# Autodesk Inventor assembly: PCB Stack Concept V03 01
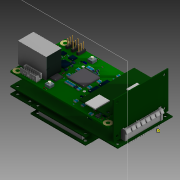
[picture p0: Inventor's stored thumbnail of the model, 180x180]
Saved by Autodesk Inventor 2013 (Build 170138000, 138)
## iProperties
Created: 2014-04-13
Part Number: PCB Stack Concept V03 01
Document SubType Name: Assembly
Designer: spichelh
Author: spichelh
## Documents named in this file (30)
- C:\Users\spichelh\Documents\GitHub\beta-hardware\Enclosure\Version 002\PCB Stack Concept V03 01.iam
- C:\Users\spichelh\Documents\GitHub\beta-hardware\Enclosure\Version 002\Enclosure-Backplate01.ipt
- C:\Users\spichelh\Documents\GitHub\beta-hardware\Enclosure\Version 002\KAC12040.ipt
- C:\Users\spichelh\Documents\GitHub\beta-hardware\Enclosure\Version 002\IRGlass.ipt
- C:\Users\spichelh\Documents\GitHub\beta-hardware\Enclosure\Version 002\Cooler.ipt
- C:\Users\spichelh\Documents\GitHub\beta-hardware\Enclosure\Version 002\Nikon Mount 02.ipt
- C:\Users\spichelh\Documents\GitHub\beta-hardware\Enclosure\Version 002\IOModulePlate01.ipt
- C:\Users\spichelh\Documents\GitHub\beta-hardware\Enclosure\Version 002\PCBModuleLeft01.ipt
- C:\Users\spichelh\Documents\GitHub\beta-hardware\Enclosure\Version 002\IOModulePlate02.ipt
- C:\Users\spichelh\Documents\GitHub\beta-hardware\Enclosure\Version 002\IOModulePlate03.ipt
- C:\Users\spichelh\Documents\GitHub\beta-hardware\Enclosure\Version 002\PCBModuleRight01.ipt
- C:\Users\spichelh\Documents\GitHub\beta-hardware\Enclosure\Version 002\LensBase02.ipt
- C:\Users\spichelh\Documents\GitHub\beta-hardware\Enclosure\Version 002\HexSaver01.ipt
- C:\Users\spichelh\Documents\GitHub\beta-hardware\Enclosure\Version 002\Enclosure03.ipt
- C:\Users\spichelh\Documents\Inventor\Content Center Files\R2013\en-US\ANSI B18.3.1M(1)\ANSI B18.3.1M - M2,5x0,45 x 16(2).ipt
- C:\Users\spichelh\Documents\Inventor\Content Center Files\R2013\en-US\ANSI B18.3.1M(1)\ANSI B18.3.1M - M2,5x0,45 x 35(2).ipt
- C:\Users\spichelh\Documents\GitHub\beta-hardware\Enclosure\Version 002\LensBaseTop01.ipt
- C:\Users\spichelh\Documents\Inventor\Content Center Files\R2013\en-US\ANSI B18.6.3(00)\ANSI B18.6.3 - 3-48 UNC - 0,25(32).ipt
- C:\Users\spichelh\Documents\GitHub\beta-hardware\Enclosure\Version 002\Unmate01.ipt
- C:\Users\spichelh\Documents\GitHub\beta-hardware\Enclosure\Version 002\Parallella.ipt
- C:\Users\spichelh\Documents\GitHub\beta-hardware\Enclosure\Version 002\SFE-Host01.ipt
- C:\Users\spichelh\Documents\GitHub\beta-hardware\Enclosure\Version 002\SFE-ProcessingBoard01.ipt
- C:\Users\spichelh\Documents\GitHub\beta-hardware\Enclosure\Version 002\CMV12000.ipt
- C:\Users\spichelh\Documents\GitHub\beta-hardware\Enclosure\Version 002\Enclosure-Backplate-Variant02.ipt
- C:\Users\spichelh\Documents\GitHub\beta-hardware\Enclosure\Version 002\PCBModuleLeft02.ipt
- C:\Users\spichelh\Documents\GitHub\beta-hardware\Enclosure\Version 002\BetaBoard01.ipt
- C:\Users\spichelh\Documents\GitHub\beta-hardware\Enclosure\Version 002\Imported Components\Zynq_Z010_uZed_F_Prod\Zynq_Z010_uZed_F_Prod.ipt
- C:\Users\spichelh\Documents\GitHub\beta-hardware\Enclosure\Version 002\Imported Components\c-5-1612163-2-h-3d\c-5-1612163-2-h-3d.ipt
- C:\Users\spichelh\Documents\GitHub\beta-hardware\Enclosure\Version 002\HidhSpeedIOShield01.ipt
- C:\Users\spichelh\Documents\GitHub\beta-hardware\Enclosure\Version 002\AddonPCB01.ipt
## Components (42 placed, 29 different names)
1. Enclosure03:1 — Flush:26, Mate:33, Mate:34, Mate:38, Flush:40, Mate:39, Insert:9, Insert:10, Insert:11, Insert:13, Insert:14, Insert:27, Insert:28, Insert:29, Mate:70, Mate:71, Flush:46, Flush:47
2. Enclosure-Backplate01:1 — Mate:38, Flush:40, Mate:75
3. KAC12040:1 — Mate:72
4. IRGlass:1 — Mate:50, Mate:51, Mate:52
5. Cooler:1 — Mate:35, Flush:43, Flush:44, Mate:67, Mate:68, Mate:69
6. Nikon Mount 02:1 — Mate:31, Mate:32, Insert:3, Mate:50, Mate:51, Mate:52, Insert:18, Insert:19, Insert:20, Insert:21
7. LensBase02:1 — Mate:31, Mate:32, Flush:26, Mate:33, Mate:34, Insert:3, Mate:35, Flush:43, Flush:44, Flush:45
8. IOModulePlate01:1 — Insert:13, Insert:14
9. PCBModuleLeft01:1
10. PCBModuleRight01:1
11. IOModulePlate02:1 — Insert:11
12. IOModulePlate03:1 — Insert:9, Insert:10
13. HexSaver01:1
14. HexSaver01:2
15. HexSaver01:3
16. HexSaver01:4
17. Broached Socket Head Cap Screw - Metric M2,5x0,45 x 16:1 — Insert:18
18. Broached Socket Head Cap Screw - Metric M2,5x0,45 x 16:2 — Insert:19
19. Broached Socket Head Cap Screw - Metric M2,5x0,45 x 16:3 — Insert:20
20. Broached Socket Head Cap Screw - Metric M2,5x0,45 x 16:4 — Insert:21
21. LensBaseTop01:1 — Flush:45, Mate:53, Mate:54, Mate:67, Mate:68, Mate:69
22. Cross Recessed 100° Flat Countersunk Head Machine Screw - Type I - Inch 3-48 UNC x 0,25:2 — Mate:53
23. Cross Recessed 100° Flat Countersunk Head Machine Screw - Type I - Inch 3-48 UNC x 0,25:1 — Mate:54
24. Broached Socket Head Cap Screw - Metric M2,5x0,45 x 35:5 — Mate:55, Mate:70, Mate:71
25. Broached Socket Head Cap Screw - Metric M2,5x0,45 x 35:6 — Insert:27, Mate:59
26. Broached Socket Head Cap Screw - Metric M2,5x0,45 x 35:7 — Insert:28, Mate:66
27. Broached Socket Head Cap Screw - Metric M2,5x0,45 x 35:8 — Insert:29, Mate:57
28. Unmate01:1 — Mate:55
29. Unmate01:2 — Mate:57
30. Unmate01:3 — Mate:59
31. Unmate01:4 — Mate:66
32. Parallella:1
33. SFE-Host01:1 — Mate:72, Mate:73, Flush:48, Flush:49, Mate:76, Flush:50, Flush:51, Flush:78
34. SFE-ProcessingBoard01:1 — Mate:73, Flush:48, Flush:49, Mate:77, Flush:85
35. CMV12000:1 — Mate:76, Flush:50, Flush:51
36. Enclosure-Backplate-Variant02:1 — Mate:75, Flush:46, Flush:47
37. PCBModuleLeft02:1 — Flush:52, Flush:79, Mate:79
38. BetaBoard01:1 — Mate:77, Flush:52, Flush:78, Flush:79, Mate:78, Flush:82, Flush:83, Mate:79, Flush:85, Flush:86, Flush:87, Mate:80, Flush:88
39. Zynq_Z010_uZed_F_Prod:1 — Flush:86, Flush:87, Mate:80, Flush:91, Mate:83, Flush:92
40. c-5-1612163-2-h-3d:1 — Mate:78, Flush:82, Flush:83, Mate:81, Mate:82
41. HidhSpeedIOShield01:1 — Mate:81, Flush:88, Mate:82
42. AddonPCB01:1 — Flush:91, Mate:83, Flush:92
## Relationships (67: Mate 32, Flush 22, Insert 13)
- Mate:31: Nikon Mount 02:1 ↔ LensBase02:1
- Mate:32: Nikon Mount 02:1 ↔ LensBase02:1
- Flush:26: Enclosure03:1 ↔ LensBase02:1
- Mate:33: Enclosure03:1 ↔ LensBase02:1
- Mate:34: Enclosure03:1 ↔ LensBase02:1
- Insert:3: Nikon Mount 02:1 ↔ LensBase02:1
- Mate:35: Cooler:1 ↔ LensBase02:1
- Mate:38 (3 mm): Enclosure03:1 ↔ Enclosure-Backplate01:1
- Flush:40: Enclosure03:1 ↔ Enclosure-Backplate01:1
- Mate:39: Enclosure03:1
- Insert:9: Enclosure03:1 ↔ IOModulePlate03:1
- Insert:10: Enclosure03:1 ↔ IOModulePlate03:1
- Insert:11: Enclosure03:1 ↔ IOModulePlate02:1
- Insert:13: Enclosure03:1 ↔ IOModulePlate01:1
- Insert:14: Enclosure03:1 ↔ IOModulePlate01:1
- Mate:50: IRGlass:1 ↔ Nikon Mount 02:1
- Mate:51 (0.5 mm): IRGlass:1 ↔ Nikon Mount 02:1
- Mate:52 (0.5 mm): IRGlass:1 ↔ Nikon Mount 02:1
- Flush:43: Cooler:1 ↔ LensBase02:1
- Flush:44: Cooler:1 ↔ LensBase02:1
- Flush:45: LensBase02:1 ↔ LensBaseTop01:1
- Mate:55: Broached Socket Head Cap Screw - Metric M2,5x0,45 x 35:5 ↔ Unmate01:1
- Mate:57: Broached Socket Head Cap Screw - Metric M2,5x0,45 x 35:8 ↔ Unmate01:2
- Mate:59: Broached Socket Head Cap Screw - Metric M2,5x0,45 x 35:6 ↔ Unmate01:3
- Mate:66: Broached Socket Head Cap Screw - Metric M2,5x0,45 x 35:7 ↔ Unmate01:4
- Mate:67: Cooler:1 ↔ LensBaseTop01:1
- Mate:68: Cooler:1 ↔ LensBaseTop01:1
- Mate:69: Cooler:1 ↔ LensBaseTop01:1
- Mate:70: Enclosure03:1 ↔ Broached Socket Head Cap Screw - Metric M2,5x0,45 x 35:5
- Mate:71: Enclosure03:1 ↔ Broached Socket Head Cap Screw - Metric M2,5x0,45 x 35:5
- Mate:72: KAC12040:1 ↔ SFE-Host01:1
- Mate:73: SFE-Host01:1 ↔ SFE-ProcessingBoard01:1
- Mate:75 (10 mm): Enclosure-Backplate01:1 ↔ Enclosure-Backplate-Variant02:1
- Flush:46: Enclosure03:1 ↔ Enclosure-Backplate-Variant02:1
- Flush:47: Enclosure03:1 ↔ Enclosure-Backplate-Variant02:1
- Flush:48: SFE-Host01:1 ↔ SFE-ProcessingBoard01:1
- Flush:49: SFE-Host01:1 ↔ SFE-ProcessingBoard01:1
- Mate:76 (3 mm): SFE-Host01:1 ↔ CMV12000:1
- Flush:50 (5 mm): SFE-Host01:1 ↔ CMV12000:1
- Flush:51 (11.75 mm): SFE-Host01:1 ↔ CMV12000:1
- Mate:77: SFE-ProcessingBoard01:1 ↔ BetaBoard01:1
- Flush:52: PCBModuleLeft02:1 ↔ BetaBoard01:1
- Flush:78: SFE-Host01:1 ↔ BetaBoard01:1
- Flush:79: PCBModuleLeft02:1 ↔ BetaBoard01:1
- Mate:78: BetaBoard01:1 ↔ c-5-1612163-2-h-3d:1
- Flush:82 (8.5 mm): BetaBoard01:1 ↔ c-5-1612163-2-h-3d:1
- Flush:83 (2 mm): BetaBoard01:1 ↔ c-5-1612163-2-h-3d:1
- Mate:79 (6 mm): PCBModuleLeft02:1 ↔ BetaBoard01:1
- Flush:85 (-21 mm): SFE-ProcessingBoard01:1 ↔ BetaBoard01:1
- Flush:86: BetaBoard01:1 ↔ Zynq_Z010_uZed_F_Prod:1
- Flush:87: BetaBoard01:1 ↔ Zynq_Z010_uZed_F_Prod:1
- Mate:80 (12 mm): BetaBoard01:1 ↔ Zynq_Z010_uZed_F_Prod:1
- Mate:81: c-5-1612163-2-h-3d:1 ↔ HidhSpeedIOShield01:1
- Flush:88: BetaBoard01:1 ↔ HidhSpeedIOShield01:1
- Mate:82: c-5-1612163-2-h-3d:1 ↔ HidhSpeedIOShield01:1
- Flush:91: Zynq_Z010_uZed_F_Prod:1 ↔ AddonPCB01:1
- Mate:83: Zynq_Z010_uZed_F_Prod:1 ↔ AddonPCB01:1
- Flush:92: Zynq_Z010_uZed_F_Prod:1 ↔ AddonPCB01:1
- Insert:18: Nikon Mount 02:1 ↔ Broached Socket Head Cap Screw - Metric M2,5x0,45 x 16:1
- Insert:19: Nikon Mount 02:1 ↔ Broached Socket Head Cap Screw - Metric M2,5x0,45 x 16:2
- Insert:20: Nikon Mount 02:1 ↔ Broached Socket Head Cap Screw - Metric M2,5x0,45 x 16:3
- Insert:21: Nikon Mount 02:1 ↔ Broached Socket Head Cap Screw - Metric M2,5x0,45 x 16:4
- Mate:53: LensBaseTop01:1 ↔ Cross Recessed 100° Flat Countersunk Head Machine Screw - Type I - Inch 3-48 UNC x 0,25:2
- Mate:54: LensBaseTop01:1 ↔ Cross Recessed 100° Flat Countersunk Head Machine Screw - Type I - Inch 3-48 UNC x 0,25:1
- Insert:27: Enclosure03:1 ↔ Broached Socket Head Cap Screw - Metric M2,5x0,45 x 35:6
- Insert:28: Enclosure03:1 ↔ Broached Socket Head Cap Screw - Metric M2,5x0,45 x 35:7
- Insert:29: Enclosure03:1 ↔ Broached Socket Head Cap Screw - Metric M2,5x0,45 x 35:8
